# Autodesk Inventor assembly: SingleCrossover_PointA
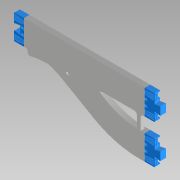
[picture p0: Inventor's stored thumbnail of the model, 180x180]
Saved by Autodesk Inventor 2021 (Build 250183000, 183)
## iProperties
Created: 2021-03-17
Part Number: SingleCrossover_PointA
Document SubType Name: Assembly
Designer: kumagai
Author: kumagai
## Documents named in this file (7)
- X:\Develop\CAD\PlaRails\Crossover\SingleCrossoverIA\SingleCrossover_PointA.iam
- X:\Develop\CAD\PlaRails\Crossover\SingleCross_PointHalf.ipt
- X:\Develop\CAD\PlaRails\RailJointFemale.ipt
- X:\Develop\CAD\PlaRails\RailJointMale.ipt
- X:\Develop\CAD\PlaRails\GlobalParameter.ipt
- X:\Develop\CAD\PlaRails\Crossover\SingleCross_CurveHalf.ipt
- X:\Develop\CAD\PlaRails\Crossover\SingleCrossoverIA.iam
## Components (5 placed, 4 different names)
1. SingleCross_PointHalf:1 — フラッシュ:1, フラッシュ:3, フラッシュ:4
2. SingleCross_CurveHalf:1 — フラッシュ:17, フラッシュ:18, フラッシュ:19
3. RailJointFemale:1 — フラッシュ:5, フラッシュ:7, フラッシュ:9
4. RailJointMale:1 — フラッシュ:11, フラッシュ:13, フラッシュ:15
5. RailJointMale:2 — フラッシュ:12, フラッシュ:14, フラッシュ:16
## Relationships (15: Flush 15)
- フラッシュ:1 [Flush]: SingleCross_PointHalf:1
- フラッシュ:3 [Flush]: SingleCross_PointHalf:1
- フラッシュ:4 [Flush]: SingleCross_PointHalf:1
- フラッシュ:5 [Flush] (-5.2 mm): RailJointFemale:1
- フラッシュ:7 [Flush] (30 mm): RailJointFemale:1
- フラッシュ:9 [Flush] (-92.5 mm): RailJointFemale:1
- フラッシュ:11 [Flush] (-5.2 mm): RailJointMale:1
- フラッシュ:12 [Flush] (-5.2 mm): RailJointMale:2
- フラッシュ:13 [Flush] (30 mm): RailJointMale:1
- フラッシュ:14 [Flush] (-30 mm): RailJointMale:2
- フラッシュ:15 [Flush] (92.5 mm): RailJointMale:1
- フラッシュ:16 [Flush] (92.5 mm): RailJointMale:2
- フラッシュ:17 [Flush]: SingleCross_CurveHalf:1
- フラッシュ:18 [Flush]: SingleCross_CurveHalf:1
- フラッシュ:19 [Flush]: SingleCross_CurveHalf:1
## Named parameters: PrinterOffset = 0 mm, StraightLength = 215 mm, RailWidth = 38 mm, OuterWall = 2 mm, InnerWall = 2.4 mm, InsideWidth = 18.6 mm, RailHeight = 8.4 mm, RailDepth = 3.2 mm, ConnectorLength = 15 mm, JointMW1 = 13 mm, JointMW2 = 9.4 mm, JointMH = 9 mm, JointFW1 = 13.3 mm, JointFW2 = 9.6 mm, JointFH = 9.5 mm, DoubleWidth = 60 mm, ViaductHeight = 66 mm, SupportGap = 0.2 mm, SupportRib = 0.5 mm
